# Autodesk Inventor assembly: XIAO-nRF52840
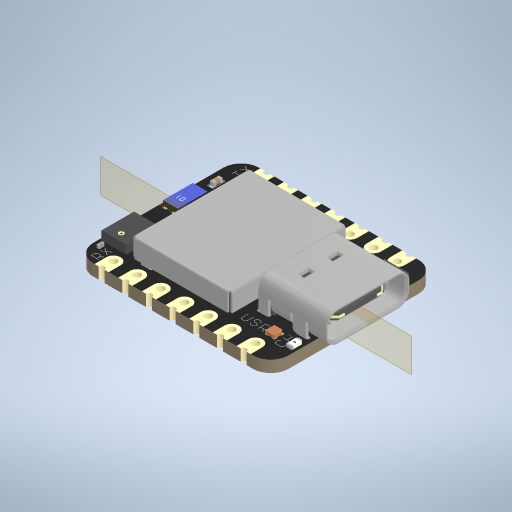
[picture p0: Inventor's stored thumbnail of the model, 512x512]
Saved by Autodesk Inventor 2024.3 (Build 283343000, 343)
## iProperties
Created: 2023-06-02
Part Number: XIAO-nRF52840
Document SubType Name: Assembly
Designer: ASUS TUF
Sending System: Autodesk Translation Framework v12.6.0.85
Preprocessor: ST-DEVELOPER v19.2
Title: XIAO-nRF52840 v15.step
## Documents named in this file (6)
- C:\Users\ASUS TUF\Documents\Inventor\ParkinsonDetection\XIAO-nRF52840 v15\XIAO-nRF52840 v15\XIAO-nRF52840 v15.iam
- C:\Users\ASUS TUF\Documents\Inventor\ParkinsonDetection\XIAO-nRF52840 v15\XIAO-nRF52840 v15\USB TYPE C PORT.iam
- C:\Users\ASUS TUF\Documents\Inventor\ParkinsonDetection\XIAO-nRF52840 v15\XIAO-nRF52840 v15\Shield.ipt
- C:\Users\ASUS TUF\Documents\Inventor\ParkinsonDetection\XIAO-nRF52840 v15\XIAO-nRF52840 v15\SKTAAAE010 v1.iam
- C:\Users\ASUS TUF\Documents\Inventor\ParkinsonDetection\XIAO-nRF52840 v15\XIAO-nRF52840 v15\PCB (1).iam
- C:\Users\ASUS TUF\Documents\Inventor\ParkinsonDetection\XIAO-nRF52840 v15\XIAO-nRF52840 v15\MSM261D3526H1CPM.iam
## Components (5 placed, 5 different names)
1. USB TYPE C PORT:1 [sub-assembly]
2. Shield:1
3. SKTAAAE010 v1:2 [sub-assembly]
4. PCB (1):1 [sub-assembly] — Flush:1
5. MSM261D3526H1CPM:1 [sub-assembly]
## Relationships (1: Flush 1)
- Flush:1 (-8.89 mm): PCB (1):1
